# Autodesk Inventor assembly: CE-8.1.1
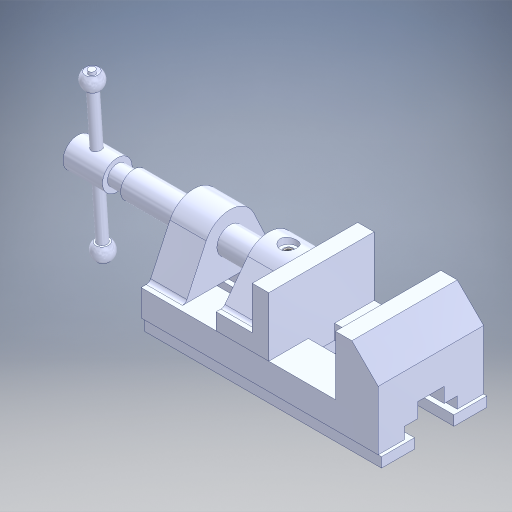
[picture p0: Inventor's stored thumbnail of the model, 512x512]
Saved by Autodesk Inventor 2024 (Build 280153000, 153)
## iProperties
Created: 2024-03-07
Part Number: CE-8.1.1
Document SubType Name: Assembly
Designer: Alex
Author: Alex
## Documents named in this file (11)
- C:\Shared\alex-bartella-schoolwork\4z03\Week 8\CE-8.1.1.iam
- C:\Shared\alex-bartella-schoolwork\4z03\Week 8\CE-8.1.1-01 STEP Files\CE-8.1.1-01-001 (Vise Body)\CE-8.1.1-01-001 (Vise Body).ipt
- C:\Shared\alex-bartella-schoolwork\4z03\Week 8\CE-8.1.1-01 STEP Files\CE-8.1.1-01-002 (Vise Jaw)\CE-8.1.1-01-002 (Vise Jaw).ipt
- C:\Shared\alex-bartella-schoolwork\4z03\Week 8\CE-8.1.1-01 STEP Files\CE-8.1.1-01-003 (Lead Screw)\CE-8.1.1-01-003 (Lead Screw).ipt
- C:\Shared\alex-bartella-schoolwork\4z03\Week 8\CE-8.1.1-01 STEP Files\CE-8.1.1-01-004 (Jaw Plate)\CE-8.1.1-01-004 (Jaw Plate).ipt
- C:\Shared\alex-bartella-schoolwork\4z03\Week 8\CE-8.1.1-01 STEP Files\CE-8.1.1-01-005 (Clamp Rails)\CE-8.1.1-01-005 (Clamp Rails).ipt
- C:\Shared\alex-bartella-schoolwork\4z03\Week 8\CE-8.1.1-01 STEP Files\CE-8.1.1-01-006 (Bar)\CE-8.1.1-01-006 (Bar).ipt
- C:\Shared\alex-bartella-schoolwork\4z03\Week 8\CE-8.1.1-01 STEP Files\CE-8.1.1-01-007 (Bar Ends)\CE-8.1.1-01-007 (Bar Ends).ipt
- C:\Users\turbo\Documents\Inventor\Content Center Files\R2024\en-US\AS 1421(2)\AS 1421 - M6 x 8 Cup Point.ipt
- C:\Users\turbo\Documents\Inventor\Content Center Files\R2024\en-US\ANSI_ASME B18.6.5M(1)\ANSI_ASME B18.6.5M - M5x0.8 x 13(1) T.ipt
- C:\Users\turbo\Documents\Inventor\Content Center Files\R2024\en-US\ANSI_ASME B18.6.5M(1)\ANSI_ASME B18.6.5M - M6x1 x 13(1) T.ipt
## Components (16 placed, 10 different names)
1. CE-8.1.1-01-001 (Vise Body):1 — Mate:1, Mate:2, Flush:1, Mate:3, Mate:4, Mate:8, Mate:9, Mate:10, Mate:11, Mate:12, Mate:13, Mate:14
2. CE-8.1.1-01-002 (Vise Jaw):1 — Mate:3, Mate:4, Mate:5, Mate:6, Mate:7, Mate:15, Rotation/Translation:1, Mate:18
3. CE-8.1.1-01-003 (Lead Screw):1 — Mate:14, Mate:15, Mate:17, Rotation/Translation:1
4. CE-8.1.1-01-004 (Jaw Plate):1 — Mate:5, Mate:6, Mate:7, Mate:23, Mate:24, Flush:6, Flush:7
5. CE-8.1.1-01-005 (Clamp Rails):1 — Mate:8, Mate:12, Mate:13, Mate:21, Mate:22, Flush:4, Flush:5
6. CE-8.1.1-01-005 (Clamp Rails):2 — Mate:9, Mate:10, Mate:11, Mate:19, Mate:20, Flush:2, Flush:3
7. CE-8.1.1-01-006 (Bar):1 — Mate:17, Insert:1, Insert:2
8. CE-8.1.1-01-007 (Bar Ends):1 — Insert:1
9. CE-8.1.1-01-007 (Bar Ends):2 — Insert:2
10. AS 1421 Cup Point - Metric M6 x 8 Cup Point:1 — Mate:18
11. Slotted Flat Countersunk Head Tapping Screw - Type T - Metric M5x0.8 x 13:1 — Mate:19, Flush:2
12. Slotted Flat Countersunk Head Tapping Screw - Type T - Metric M5x0.8 x 13:2 — Mate:20, Flush:3
13. Slotted Flat Countersunk Head Tapping Screw - Type T - Metric M5x0.8 x 13:3 — Mate:21, Flush:4
14. Slotted Flat Countersunk Head Tapping Screw - Type T - Metric M5x0.8 x 13:4 — Mate:22, Flush:5
15. Slotted Flat Countersunk Head Tapping Screw - Type T - Metric M6x1 x 13:1 — Mate:23, Flush:6, Mate:25
16. Slotted Flat Countersunk Head Tapping Screw - Type T - Metric M6x1 x 13:2 — Mate:24, Flush:7, Mate:25
## Relationships (34: Mate 24, Flush 7, Insert 2, RelateRotateTranslate 1)
- Mate:1: CE-8.1.1-01-001 (Vise Body):1
- Mate:2: CE-8.1.1-01-001 (Vise Body):1
- Flush:1: CE-8.1.1-01-001 (Vise Body):1
- Mate:3: CE-8.1.1-01-001 (Vise Body):1 ↔ CE-8.1.1-01-002 (Vise Jaw):1
- Mate:4: CE-8.1.1-01-001 (Vise Body):1 ↔ CE-8.1.1-01-002 (Vise Jaw):1
- Mate:5: CE-8.1.1-01-002 (Vise Jaw):1 ↔ CE-8.1.1-01-004 (Jaw Plate):1
- Mate:6: CE-8.1.1-01-002 (Vise Jaw):1 ↔ CE-8.1.1-01-004 (Jaw Plate):1
- Mate:7: CE-8.1.1-01-002 (Vise Jaw):1 ↔ CE-8.1.1-01-004 (Jaw Plate):1
- Mate:8: CE-8.1.1-01-001 (Vise Body):1 ↔ CE-8.1.1-01-005 (Clamp Rails):1
- Mate:9: CE-8.1.1-01-001 (Vise Body):1 ↔ CE-8.1.1-01-005 (Clamp Rails):2
- Mate:10: CE-8.1.1-01-001 (Vise Body):1 ↔ CE-8.1.1-01-005 (Clamp Rails):2
- Mate:11: CE-8.1.1-01-001 (Vise Body):1 ↔ CE-8.1.1-01-005 (Clamp Rails):2
- Mate:12: CE-8.1.1-01-001 (Vise Body):1 ↔ CE-8.1.1-01-005 (Clamp Rails):1
- Mate:13: CE-8.1.1-01-001 (Vise Body):1 ↔ CE-8.1.1-01-005 (Clamp Rails):1
- Mate:14: CE-8.1.1-01-001 (Vise Body):1 ↔ CE-8.1.1-01-003 (Lead Screw):1
- Mate:15: CE-8.1.1-01-002 (Vise Jaw):1 ↔ CE-8.1.1-01-003 (Lead Screw):1
- Mate:17: CE-8.1.1-01-003 (Lead Screw):1 ↔ CE-8.1.1-01-006 (Bar):1
- Insert:1: CE-8.1.1-01-006 (Bar):1 ↔ CE-8.1.1-01-007 (Bar Ends):1
- Insert:2: CE-8.1.1-01-006 (Bar):1 ↔ CE-8.1.1-01-007 (Bar Ends):2
- Rotation/Translation:1 [RelateRotateTranslate] (2 mm): CE-8.1.1-01-002 (Vise Jaw):1 ↔ CE-8.1.1-01-003 (Lead Screw):1
- Mate:18: CE-8.1.1-01-002 (Vise Jaw):1 ↔ AS 1421 Cup Point - Metric M6 x 8 Cup Point:1
- Mate:19: CE-8.1.1-01-005 (Clamp Rails):2 ↔ Slotted Flat Countersunk Head Tapping Screw - Type T - Metric M5x0.8 x 13:1
- Mate:20: CE-8.1.1-01-005 (Clamp Rails):2 ↔ Slotted Flat Countersunk Head Tapping Screw - Type T - Metric M5x0.8 x 13:2
- Mate:21: CE-8.1.1-01-005 (Clamp Rails):1 ↔ Slotted Flat Countersunk Head Tapping Screw - Type T - Metric M5x0.8 x 13:3
- Mate:22: CE-8.1.1-01-005 (Clamp Rails):1 ↔ Slotted Flat Countersunk Head Tapping Screw - Type T - Metric M5x0.8 x 13:4
- Flush:2: CE-8.1.1-01-005 (Clamp Rails):2 ↔ Slotted Flat Countersunk Head Tapping Screw - Type T - Metric M5x0.8 x 13:1
- Flush:3: CE-8.1.1-01-005 (Clamp Rails):2 ↔ Slotted Flat Countersunk Head Tapping Screw - Type T - Metric M5x0.8 x 13:2
- Flush:4: CE-8.1.1-01-005 (Clamp Rails):1 ↔ Slotted Flat Countersunk Head Tapping Screw - Type T - Metric M5x0.8 x 13:3
- Flush:5: CE-8.1.1-01-005 (Clamp Rails):1 ↔ Slotted Flat Countersunk Head Tapping Screw - Type T - Metric M5x0.8 x 13:4
- Mate:23: CE-8.1.1-01-004 (Jaw Plate):1 ↔ Slotted Flat Countersunk Head Tapping Screw - Type T - Metric M6x1 x 13:1
- Mate:24: CE-8.1.1-01-004 (Jaw Plate):1 ↔ Slotted Flat Countersunk Head Tapping Screw - Type T - Metric M6x1 x 13:2
- Flush:6: CE-8.1.1-01-004 (Jaw Plate):1 ↔ Slotted Flat Countersunk Head Tapping Screw - Type T - Metric M6x1 x 13:1
- Flush:7: CE-8.1.1-01-004 (Jaw Plate):1 ↔ Slotted Flat Countersunk Head Tapping Screw - Type T - Metric M6x1 x 13:2
- Mate:25: Slotted Flat Countersunk Head Tapping Screw - Type T - Metric M6x1 x 13:1 ↔ Slotted Flat Countersunk Head Tapping Screw - Type T - Metric M6x1 x 13:2
